# Autodesk Inventor assembly: 6Plaction-asm
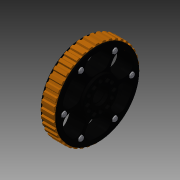
[picture p0: Inventor's stored thumbnail of the model, 180x180]
Saved by Autodesk Inventor 2013 (Build 170138000, 138)
## iProperties
Created: 2013-01-17
Part Number: 6Plaction-asm
Document SubType Name: Assembly
Designer: Moses
Mass: 367.41 g
Surface Area: 1270.02 cm^2
Volume: 321.023 cm^3
Author: Moses
## Documents named in this file (5)
- C:\Users\Moses\Documents\GitHub\frc2013CAD\Drivetrain\6Plaction-asm\6Plaction-asm.iam
- C:\Users\Moses\Documents\GitHub\frc2013CAD\Drivetrain\6Plaction-asm\6MW_d01.ipt
- C:\Users\Moses\Documents\GitHub\frc2013CAD\Drivetrain\6Plaction-asm\10-32x1000shcs.ipt
- C:\Users\Moses\Documents\GitHub\frc2013CAD\Drivetrain\6Plaction-asm\10-32_locknut.ipt
- C:\Users\Moses\Documents\GitHub\frc2013CAD\Drivetrain\6Plaction-asm\6plactiontread.ipt
## Components (15 placed, 4 different names)
1. 6MW_d01:1 — Mate:2
2. 6MW_d01:2 — Mate:1
3. 10-32x1000shcs:1
4. 10-32x1000shcs:2
5. 10-32x1000shcs:3
6. 10-32x1000shcs:4
7. 10-32x1000shcs:5
8. 10-32x1000shcs:6
9. 10-32_locknut:1
10. 10-32_locknut:2
11. 10-32_locknut:3
12. 10-32_locknut:4
13. 10-32_locknut:5
14. 10-32_locknut:6
15. 6plactiontread:1 — Mate:1, Mate:2
## Relationships (2: Mate 2)
- Mate:1: 6MW_d01:2 ↔ 6plactiontread:1
- Mate:2: 6MW_d01:1 ↔ 6plactiontread:1
